# Autodesk Inventor assembly: Assem1
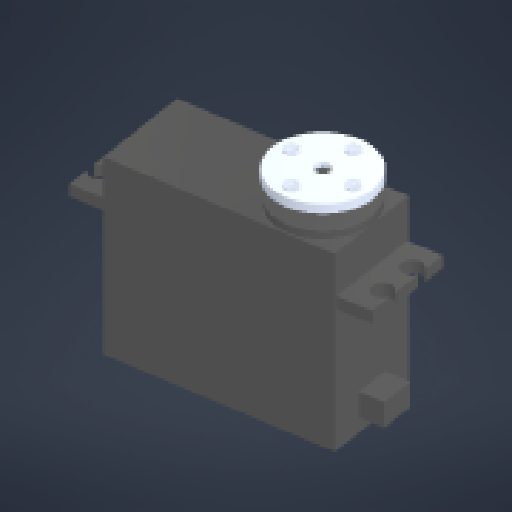
[picture p0: Inventor's stored thumbnail of the model, 512x512]
Saved by Autodesk Inventor 2027.1 (Build 311270010, 270A)
## iProperties
Created: 2021-09-09
Part Number: Assem1
Document SubType Name: Assembly
Designer: daniel
Sending System: SOLIDWORKS 2020
Last Saved Date: 2021-09-09
last saved by: DIMA
Author: daniel
## Documents named in this file (3)
- C:\Users\danda\Downloads\standard-servo-motor-black-1.snapshot.7\Assem1\Assem1.iam
- C:\Users\danda\Downloads\standard-servo-motor-black-1.snapshot.7\Assem1\body.ipt
- C:\Users\danda\Downloads\mg995-servo-motor-metal-horn-1.snapshot.2\servo horn\servo horn.ipt
## Components (2 placed, 2 different names)
1. body-1 — Mate:1, Mate:2
2. servo horn:1 — Mate:1, Mate:2
## Relationships (2: Mate 2)
- Mate:1: body-1 ↔ servo horn:1
- Mate:2: body-1 ↔ servo horn:1
